# Autodesk Inventor assembly: 車軸受け
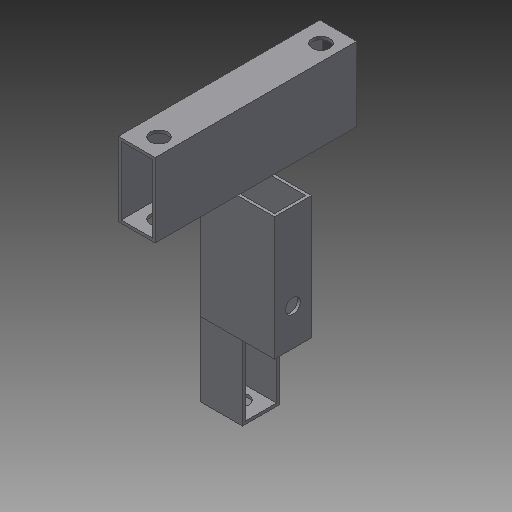
[picture p0: Inventor's stored thumbnail of the model, 512x512]
Saved by Autodesk Inventor 2018 (Build 220112000, 112)
## iProperties
Created: 2017-09-15
Part Number: 車軸受け
Material: 一般
Document SubType Name: Assembly
Designer: mura5
Author: mura5
## Documents named in this file (4)
- C:\Users\mura5\Documents\RBBR\cart\前足改\車軸受け改改\車軸受け_後.iam
- C:\Users\mura5\Documents\RBBR\cart\前足改\車軸受け改改\車軸受け1.ipt
- C:\Users\mura5\Documents\RBBR\cart\前足改\車軸受け改改\車軸受け2.ipt
- C:\Users\mura5\Documents\RBBR\cart\前足改\車軸受け改改\車軸受け3.ipt
## Components (3 placed, 3 different names)
1. 車軸受け1:1 — リジッド:2, フラッシュ:1, メイト:1, フラッシュ:2
2. 車軸受け3:1 — フラッシュ:1, メイト:1, フラッシュ:2
3. 車軸受け2:2 — リジッド:2
## Relationships (4: Flush 2, WeldJoint 1, Mate 1)
- リジッド:2 [WeldJoint]: 車軸受け1:1 ↔ 車軸受け2:2
- フラッシュ:1 [Flush]: 車軸受け1:1 ↔ 車軸受け3:1
- メイト:1 [Mate]: 車軸受け1:1 ↔ 車軸受け3:1
- フラッシュ:2 [Flush] (66.75 mm): 車軸受け1:1 ↔ 車軸受け3:1
